# Autodesk Inventor assembly: A2017_T5_02
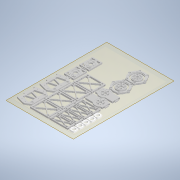
[picture p0: Inventor's stored thumbnail of the model, 180x180]
Saved by Autodesk Inventor 2020 (Build 240168000, 168)
## iProperties
Created: 2021-08-27
Part Number: A2017_T5_02
Document SubType Name: Assembly
Designer: Masato
Author: Masato
## Documents named in this file (10)
- C:\Users\naoki\Documents\Inventor\CitBrains\git_clone\SUSTAINA_ver1_0\GFRP_2\SUSTAINA-OP\Cam\A2017_T5_02.iam
- C:\Users\naoki\Documents\Inventor\CitBrains\git_clone\SUSTAINA_ver1_0\GFRP_2\SUSTAINA-OP\Cam\DisposableBoard.ipt
- C:\Users\naoki\Documents\Inventor\CitBrains\git_clone\SUSTAINA_ver1_0\GFRP_2\SUSTAINA-OP\LowerBody\Knee\Knee_clamp.ipt
- C:\Users\naoki\Documents\Inventor\CitBrains\git_clone\SUSTAINA_ver1_0\GFRP_2\SUSTAINA-OP\UpperBody\Trunk\Trunk_lower_side_frame.ipt
- C:\Users\naoki\Documents\Inventor\CitBrains\git_clone\SUSTAINA_ver1_0\GFRP_2\SUSTAINA-OP\UpperBody\Arm\Shoulder_horn_frame.ipt
- C:\Users\naoki\Documents\Inventor\CitBrains\git_clone\SUSTAINA_ver1_0\GFRP_2\SUSTAINA-OP\LowerBody\Link\FrontLink_diagonal.ipt
- C:\Users\naoki\Documents\Inventor\CitBrains\git_clone\SUSTAINA_ver1_0\GFRP_2\SUSTAINA-OP\LowerBody\Link\BackLink_diagonal.ipt
- C:\Users\naoki\Documents\Inventor\CitBrains\git_clone\SUSTAINA_ver1_0\GFRP_2\SUSTAINA-OP\LowerBody\Leg_joit\Leg_joint_yaw_frame.ipt
- C:\Users\naoki\Documents\Inventor\CitBrains\git_clone\SUSTAINA_ver1_0\GFRP_2\SUSTAINA-OP\UpperBody\Trunk\CrossRollerBearing\Inner_support_stand.ipt
- C:\Users\naoki\Documents\Inventor\CitBrains\git_clone\SUSTAINA_ver1_0\GFRP_2\SUSTAINA-OP\UpperBody\Trunk\CrossRollerBearing\Outer_support_stand.ipt
## Components (24 placed, 9 different names)
1. DisposableBoard:1 — メイト:2, メイト:1, フラッシュ:1, フラッシュ:2, メイト:4, メイト:5, メイト:6, メイト:7, メイト:8, フラッシュ:4, フラッシュ:7, 正接:1, 角度:1, フラッシュ:8, 正接:2, メイト:13, メイト:14, メイト:15, メイト:18, メイト:19, メイト:20, メイト:21, 角度:2, 角度:3, 角度:4, 角度:5
2. Shoulder_horn_frame:1 — メイト:8, メイト:17, フラッシュ:11, 正接:6, 正接:13, メイト:22
3. Shoulder_horn_frame:2 — メイト:13, メイト:17, フラッシュ:11
4. Leg_joint_yaw_frame:1 — メイト:15, フラッシュ:9, 正接:5, 正接:7, 正接:9, 正接:10
5. Leg_joint_yaw_frame:2 — メイト:14, メイト:16, フラッシュ:9, 正接:4, 正接:5
6. Inner_support_stand:1 — メイト:21, 正接:11, 角度:4
7. Inner_support_stand:2 — メイト:18, 正接:12, 角度:5
8. Outer_support_stand:1 — メイト:20, 角度:3, 正接:8, 正接:10, 正接:12
9. Outer_support_stand:2 — メイト:19, 角度:2, 正接:7, 正接:8, 正接:9, 正接:11
10. FrontLink_diagonal:1 — メイト:6, フラッシュ:4, メイト:10, メイト:12
11. FrontLink_diagonal:2
12. FrontLink_diagonal:3 — メイト:16
13. FrontLink_diagonal:4 — メイト:22
14. BackLink_diagonal:1 — メイト:5, メイト:10, フラッシュ:7, 正接:3
15. BackLink_diagonal:2
16. BackLink_diagonal:3
17. BackLink_diagonal:4 — 正接:4
18. Trunk_lower_side_frame:1 — メイト:4, メイト:12, 正接:1, フラッシュ:8
19. Trunk_lower_side_frame:2 — 正接:6, 正接:13
20. Knee_clamp:1 — メイト:7, 角度:1, 正接:2, 正接:3
21. Knee_clamp:2
22. Knee_clamp:3
23. Knee_clamp:4
24. Knee_clamp:5
## Component patterns: (4 elements, first: FrontLink_diagonal:1), (4 elements, first: BackLink_diagonal:1), (2 elements, first: Trunk_lower_side_frame:1), (5 elements, first: Knee_clamp:1)
## Relationships (44: Mate 19, Tangent 13, Flush 7, Angle 5)
- メイト:2 [Mate]: DisposableBoard:1
- メイト:1 [Mate]: DisposableBoard:1
- フラッシュ:1 [Flush]: DisposableBoard:1
- フラッシュ:2 [Flush]: DisposableBoard:1
- メイト:4 [Mate]: DisposableBoard:1 ↔ Trunk_lower_side_frame:1
- メイト:5 [Mate]: DisposableBoard:1 ↔ BackLink_diagonal:1
- メイト:6 [Mate]: DisposableBoard:1 ↔ FrontLink_diagonal:1
- メイト:7 [Mate]: DisposableBoard:1 ↔ Knee_clamp:1
- メイト:8 [Mate]: DisposableBoard:1 ↔ Shoulder_horn_frame:1
- フラッシュ:4 [Flush] (2 mm): DisposableBoard:1 ↔ FrontLink_diagonal:1
- メイト:10 [Mate] (2.5 mm): FrontLink_diagonal:1 ↔ BackLink_diagonal:1
- フラッシュ:7 [Flush] (2 mm): DisposableBoard:1 ↔ BackLink_diagonal:1
- メイト:12 [Mate] (2.5 mm): FrontLink_diagonal:1 ↔ Trunk_lower_side_frame:1
- 正接:1 [Tangent] (2 mm): DisposableBoard:1 ↔ Trunk_lower_side_frame:1
- 角度:1 [Angle] (45 deg): DisposableBoard:1 ↔ Knee_clamp:1
- フラッシュ:8 [Flush] (2 mm): DisposableBoard:1 ↔ Trunk_lower_side_frame:1
- 正接:2 [Tangent] (2 mm): DisposableBoard:1 ↔ Knee_clamp:1
- 正接:3 [Tangent] (3.4 mm): BackLink_diagonal:1 ↔ Knee_clamp:1
- メイト:13 [Mate]: DisposableBoard:1 ↔ Shoulder_horn_frame:2
- メイト:14 [Mate]: DisposableBoard:1 ↔ Leg_joint_yaw_frame:2
- メイト:15 [Mate]: DisposableBoard:1 ↔ Leg_joint_yaw_frame:1
- メイト:16 [Mate] (2.5 mm): Leg_joint_yaw_frame:2 ↔ FrontLink_diagonal:3
- フラッシュ:9 [Flush]: Leg_joint_yaw_frame:1 ↔ Leg_joint_yaw_frame:2
- 正接:4 [Tangent] (2.5 mm): Leg_joint_yaw_frame:2 ↔ BackLink_diagonal:4
- 正接:5 [Tangent] (3 mm): Leg_joint_yaw_frame:1 ↔ Leg_joint_yaw_frame:2
- メイト:17 [Mate] (2.5 mm): Shoulder_horn_frame:1 ↔ Shoulder_horn_frame:2
- フラッシュ:11 [Flush]: Shoulder_horn_frame:1 ↔ Shoulder_horn_frame:2
- メイト:18 [Mate]: DisposableBoard:1 ↔ Inner_support_stand:2
- メイト:19 [Mate]: DisposableBoard:1 ↔ Outer_support_stand:2
- メイト:20 [Mate]: DisposableBoard:1 ↔ Outer_support_stand:1
- メイト:21 [Mate]: DisposableBoard:1 ↔ Inner_support_stand:1
- 正接:6 [Tangent] (2.5 mm): Shoulder_horn_frame:1 ↔ Trunk_lower_side_frame:2
- 角度:2 [Angle] (30 deg): DisposableBoard:1 ↔ Outer_support_stand:2
- 角度:3 [Angle] (30 deg): DisposableBoard:1 ↔ Outer_support_stand:1
- 正接:7 [Tangent] (2.5 mm): Leg_joint_yaw_frame:1 ↔ Outer_support_stand:2
- 正接:8 [Tangent] (2.5 mm): Outer_support_stand:1 ↔ Outer_support_stand:2
- 正接:9 [Tangent]: Leg_joint_yaw_frame:1 ↔ Outer_support_stand:2
- 正接:10 [Tangent]: Leg_joint_yaw_frame:1 ↔ Outer_support_stand:1
- 正接:11 [Tangent] (-4 mm): Inner_support_stand:1 ↔ Outer_support_stand:2
- 正接:12 [Tangent] (-4 mm): Inner_support_stand:2 ↔ Outer_support_stand:1
- 角度:4 [Angle] (0 deg): DisposableBoard:1 ↔ Inner_support_stand:1
- 角度:5 [Angle] (0 deg): DisposableBoard:1 ↔ Inner_support_stand:2
- 正接:13 [Tangent] (2.5 mm): Shoulder_horn_frame:1 ↔ Trunk_lower_side_frame:2
- メイト:22 [Mate] (6.9 mm): Shoulder_horn_frame:1 ↔ FrontLink_diagonal:4
